# Autodesk Inventor assembly: Bearing_Support
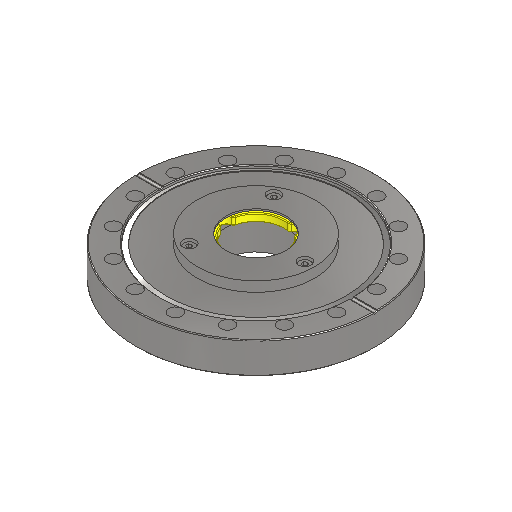
[picture p0: Inventor's stored thumbnail of the model, 512x512]
Saved by Autodesk Inventor 2026.2 (Build 302298000, 298)
## iProperties
Created: 2026-07-16
Part Number: Bearing_Support
Document SubType Name: Assembly
Designer: zetsu
Author: zetsu
## Documents named in this file (5)
- D:\repos\PIHTI\Plasma Vessel_2026\Bearing_Support.iam
- D:\repos\PIHTI\Plasma Vessel_2026\contents\CF_152-70_bearing_1.ipt
- D:\repos\PIHTI\Plasma Vessel_2026\contents\clamp_for_bearing.ipt
- D:\repos\PIHTI\Plasma Vessel_2026\contents\B_probe_bearing_clamp.ipt
- D:\repos\PIHTI\Plasma Vessel_2026\contents\M4×8-VentedHexSocket.ipt
## Components (6 placed, 4 different names)
1. CF_152-70_bearing_1:1 — メイト:1, メイト:2, メイト:3, メイト:4, メイト:5
2. clamp_for_bearing:1 — メイト:3, メイト:4, メイト:5, メイト:6, メイト:7, メイト:8, メイト:9, メイト:10, メイト:11
3. B_probe_bearing_clamp:1 — メイト:1, メイト:2
4. M4×8-VentedHexSocket:1 — メイト:6, メイト:7
5. M4×8-VentedHexSocket:2 — メイト:8, メイト:9
6. M4×8-VentedHexSocket:3 — メイト:10, メイト:11
## Relationships (11: Mate 11)
- メイト:1 [Mate]: CF_152-70_bearing_1:1 ↔ B_probe_bearing_clamp:1
- メイト:2 [Mate]: CF_152-70_bearing_1:1 ↔ B_probe_bearing_clamp:1
- メイト:3 [Mate]: CF_152-70_bearing_1:1 ↔ clamp_for_bearing:1
- メイト:4 [Mate]: CF_152-70_bearing_1:1 ↔ clamp_for_bearing:1
- メイト:5 [Mate]: CF_152-70_bearing_1:1 ↔ clamp_for_bearing:1
- メイト:6 [Mate]: clamp_for_bearing:1 ↔ M4×8-VentedHexSocket:1
- メイト:7 [Mate]: clamp_for_bearing:1 ↔ M4×8-VentedHexSocket:1
- メイト:8 [Mate]: clamp_for_bearing:1 ↔ M4×8-VentedHexSocket:2
- メイト:9 [Mate]: clamp_for_bearing:1 ↔ M4×8-VentedHexSocket:2
- メイト:10 [Mate]: clamp_for_bearing:1 ↔ M4×8-VentedHexSocket:3
- メイト:11 [Mate]: clamp_for_bearing:1 ↔ M4×8-VentedHexSocket:3
